# Autodesk Inventor assembly: 00_005_TIBIA_R1
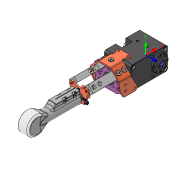
[picture p0: Inventor's stored thumbnail of the model, 180x180]
Saved by Autodesk Inventor 2021.2 (Build 252289000, 289)
## iProperties
Created: 2018-02-01
Part Number: 00_005_TIBIA_R1
Material: 一般
Document SubType Name: Assembly
Designer: y6tada
Mass: 98.3533 g
Surface Area: 375.997 cm^2
Volume: 64.3806 cm^3
Density: 1.52768 g/cm^3
Author: y6tada
## Documents named in this file (13)
- C:\Workspace\HaptHexa\Hardware\Inventor\00_005_TIBIA_R1.iam
- C:\Workspace\HaptHexa\Hardware\Inventor\11_019_TIBIA_CFRP_PIPE_R1.ipt
- C:\Workspace\HaptHexa\Hardware\Inventor\16_024_LOAD_CELL_MOUNT_BRACKET_R1.ipt
- C:\Workspace\HaptHexa\Hardware\Inventor\20_020_LOAD_CELL_R2.ipt
- C:\Workspace\HaptHexa\Hardware\Inventor\16_030_TIBIA_SENSOR_BASE_R1.ipt
- C:\Workspace\HaptHexa\Hardware\Inventor\16_021_COUPLER_BASE_R1.ipt
- C:\Workspace\HaptHexa\Hardware\Inventor\16_023_LOAD_CELL_CONTACT_PIN_R1.ipt
- C:\Workspace\HaptHexa\Hardware\Inventor\00_015_FORCE_SENSOR_AMP_R1.iam
- C:\Workspace\HaptHexa\Hardware\Inventor\00_025_SHOE_R1.iam
- C:\Workspace\HaptHexa\Hardware\Inventor\20_001_DYNAMIXEL_X430_R1.ipt
- C:\Workspace\HaptHexa\Hardware\Inventor\16_029_X430_FREE_HORN_R1.ipt
- C:\Workspace\HaptHexa\Hardware\Inventor\10_051_LOW_HEAD_CAP_BOLT_M3X6_R1.ipt
- C:\Workspace\HaptHexa\Hardware\Inventor\00_052_LOADCELL_CONTACT_R1.iam
## Components (18 placed, 12 different names)
1. LEG_PIPE_CFRP_SHORT:1 — メイト:46, メイト:47, メイト:59, Flush:65, フラッシュ:64, メイト:63
2. 16_024_LOAD_CELL_MOUNT_BRACKET_R1:1 — メイト:34, メイト:35, メイト:36, メイト:37, メイト:38, メイト:39, メイト:48, メイト:49, Mate:64, Mate:65, Mate:66, Insert:2, Insert:3, Insert:4, Insert:5, Insert:6
3. 20_020_LOAD_CELL_R2:1 — メイト:34, メイト:35, メイト:36, メイト:55, フラッシュ:4
4. 20_020_LOAD_CELL_R2:2 — メイト:37, メイト:38, メイト:39, メイト:56, フラッシュ:5
5. 16_030_TIBIA_SENSOR_BASE_R1:1 — メイト:48, メイト:49, メイト:50, メイト:51, メイト:53, メイト:57, メイト:58, 角度:3
6. 16_021_COUPLER_BASE_R1:1 — メイト:46, メイト:47, メイト:50, メイト:51, メイト:53
7. 16_023_LOAD_CELL_CONTACT_PIN_R1:1 — メイト:55, フラッシュ:4
8. 16_023_LOAD_CELL_CONTACT_PIN_R1:2 — メイト:56, フラッシュ:5
9. 00_015_FORCE_SENSOR_AMP_R1:1 [sub-assembly] — メイト:57, メイト:58, 角度:3
10. 00_025_SHOE_R1:1 [sub-assembly] — メイト:59, Flush:65, メイト:63
11. 20_001_DYNAMIXEL_X430_R1:1 — Mate:64, Mate:65, Mate:66, Insert:1
12. 16_029_X430_FREE_HORN_R1:1 — Insert:1
13. 10_051_LOW_HEAD_CAP_BOLT_M3X6_R1:1 — Insert:2
14. 10_051_LOW_HEAD_CAP_BOLT_M3X6_R1:2 — Insert:3
15. 10_051_LOW_HEAD_CAP_BOLT_M3X6_R1:3 — Insert:4
16. 10_051_LOW_HEAD_CAP_BOLT_M3X6_R1:4 — Insert:5
17. 00_052_LOADCELL_CONTACT_R1:1 [sub-assembly]
18. 10_051_LOW_HEAD_CAP_BOLT_M3X6_R1:5 — Insert:6
## Relationships (37: Mate 25, Insert 6, Flush 5, Angle 1)
- メイト:34 [Mate]: 16_024_LOAD_CELL_MOUNT_BRACKET_R1:1 ↔ 20_020_LOAD_CELL_R2:1
- メイト:35 [Mate]: 16_024_LOAD_CELL_MOUNT_BRACKET_R1:1 ↔ 20_020_LOAD_CELL_R2:1
- メイト:36 [Mate]: 16_024_LOAD_CELL_MOUNT_BRACKET_R1:1 ↔ 20_020_LOAD_CELL_R2:1
- メイト:37 [Mate]: 16_024_LOAD_CELL_MOUNT_BRACKET_R1:1 ↔ 20_020_LOAD_CELL_R2:2
- メイト:38 [Mate]: 16_024_LOAD_CELL_MOUNT_BRACKET_R1:1 ↔ 20_020_LOAD_CELL_R2:2
- メイト:39 [Mate]: 16_024_LOAD_CELL_MOUNT_BRACKET_R1:1 ↔ 20_020_LOAD_CELL_R2:2
- [Mate]: LEG_PIPE_CFRP_SHORT:1 ↔ 00_052_LOADCELL_CONTACT_R1:1
- [Flush] (-1 mm): 20_020_LOAD_CELL_R2:1 ↔ 00_052_LOADCELL_CONTACT_R1:1
- [Mate]: LEG_PIPE_CFRP_SHORT:1 ↔ 00_052_LOADCELL_CONTACT_R1:1
- メイト:46 [Mate]: LEG_PIPE_CFRP_SHORT:1 ↔ 16_021_COUPLER_BASE_R1:1
- メイト:47 [Mate]: LEG_PIPE_CFRP_SHORT:1 ↔ 16_021_COUPLER_BASE_R1:1
- メイト:48 [Mate]: 16_024_LOAD_CELL_MOUNT_BRACKET_R1:1 ↔ 16_030_TIBIA_SENSOR_BASE_R1:1
- メイト:49 [Mate]: 16_024_LOAD_CELL_MOUNT_BRACKET_R1:1 ↔ 16_030_TIBIA_SENSOR_BASE_R1:1
- メイト:50 [Mate]: 16_030_TIBIA_SENSOR_BASE_R1:1 ↔ 16_021_COUPLER_BASE_R1:1
- メイト:51 [Mate]: 16_030_TIBIA_SENSOR_BASE_R1:1 ↔ 16_021_COUPLER_BASE_R1:1
- メイト:53 [Mate]: 16_030_TIBIA_SENSOR_BASE_R1:1 ↔ 16_021_COUPLER_BASE_R1:1
- メイト:55 [Mate]: 20_020_LOAD_CELL_R2:1 ↔ 16_023_LOAD_CELL_CONTACT_PIN_R1:1
- フラッシュ:4 [Flush] (3 mm): 20_020_LOAD_CELL_R2:1 ↔ 16_023_LOAD_CELL_CONTACT_PIN_R1:1
- メイト:56 [Mate]: 20_020_LOAD_CELL_R2:2 ↔ 16_023_LOAD_CELL_CONTACT_PIN_R1:2
- フラッシュ:5 [Flush] (3 mm): 20_020_LOAD_CELL_R2:2 ↔ 16_023_LOAD_CELL_CONTACT_PIN_R1:2
- メイト:57 [Mate]: 16_030_TIBIA_SENSOR_BASE_R1:1 ↔ 00_015_FORCE_SENSOR_AMP_R1:1
- メイト:58 [Mate]: 16_030_TIBIA_SENSOR_BASE_R1:1 ↔ 00_015_FORCE_SENSOR_AMP_R1:1
- 角度:3 [Angle] (0 deg): 16_030_TIBIA_SENSOR_BASE_R1:1 ↔ 00_015_FORCE_SENSOR_AMP_R1:1
- メイト:59 [Mate]: LEG_PIPE_CFRP_SHORT:1 ↔ 00_025_SHOE_R1:1
- Flush:65: LEG_PIPE_CFRP_SHORT:1 ↔ 00_025_SHOE_R1:1
- [Mate]: LEG_PIPE_CFRP_SHORT:1 ↔ 00_052_LOADCELL_CONTACT_R1:1
- フラッシュ:64 [Flush]: LEG_PIPE_CFRP_SHORT:1
- メイト:63 [Mate]: LEG_PIPE_CFRP_SHORT:1 ↔ 00_025_SHOE_R1:1
- Mate:64: 16_024_LOAD_CELL_MOUNT_BRACKET_R1:1 ↔ 20_001_DYNAMIXEL_X430_R1:1
- Mate:65: 16_024_LOAD_CELL_MOUNT_BRACKET_R1:1 ↔ 20_001_DYNAMIXEL_X430_R1:1
- Mate:66: 16_024_LOAD_CELL_MOUNT_BRACKET_R1:1 ↔ 20_001_DYNAMIXEL_X430_R1:1
- Insert:1: 20_001_DYNAMIXEL_X430_R1:1 ↔ 16_029_X430_FREE_HORN_R1:1
- Insert:2: 16_024_LOAD_CELL_MOUNT_BRACKET_R1:1 ↔ 10_051_LOW_HEAD_CAP_BOLT_M3X6_R1:1
- Insert:3: 16_024_LOAD_CELL_MOUNT_BRACKET_R1:1 ↔ 10_051_LOW_HEAD_CAP_BOLT_M3X6_R1:2
- Insert:4: 16_024_LOAD_CELL_MOUNT_BRACKET_R1:1 ↔ 10_051_LOW_HEAD_CAP_BOLT_M3X6_R1:3
- Insert:5: 16_024_LOAD_CELL_MOUNT_BRACKET_R1:1 ↔ 10_051_LOW_HEAD_CAP_BOLT_M3X6_R1:4
- Insert:6: 16_024_LOAD_CELL_MOUNT_BRACKET_R1:1 ↔ 10_051_LOW_HEAD_CAP_BOLT_M3X6_R1:5
## Named parameters: sa_0 = 1e-13, sa_1 = -6e-13, sa_2 = -500, sa_3 = -353.553, sa_4 = -5e-13, sa_5 = -353.553, sa_6 = -500, sa_7 = -0, sa_8 = -1e-13, sa_9 = -0, sa_10 = 500, sa_11 = -6e-13
note: some values were not read from the file. Shown as the stored number, unit unknown: "sa_0", "sa_1", "sa_2", "sa_3", "sa_4", "sa_5", "sa_6", "sa_7", "sa_8", "sa_9", "sa_10", "sa_11".
